# Autodesk Inventor assembly: Bearing Assembly
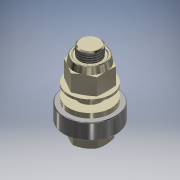
[picture p0: Inventor's stored thumbnail of the model, 180x180]
Saved by Autodesk Inventor 2018.2 (Build 222227000, 227)
## iProperties
Created: 2018-01-21
Part Number: Bearing Assembly
Document SubType Name: Assembly
Designer: torba
Author: torba
## Documents named in this file (6)
- C:\Users\torba\OneDrive\Documents\Inventor\Plasma 5x10\Bearing Assembly.iam
- C:\Users\torba\OneDrive\Documents\Inventor\Plasma 5x10\6202RS Bearing.ipt
- C:\Users\torba\OneDrive\Documents\Inventor\Content Center Files\R2018\en-US\AS 2465(2)\AS 2465 - 9_16 x 1 3_4  UNF.ipt
- C:\Users\torba\OneDrive\Documents\Inventor\Content Center Files\R2018\en-US\ANSI B18.22.1\ANSI B18.22.1 - 9_16 - narrow - Type B.ipt
- C:\Users\torba\OneDrive\Documents\Inventor\Plasma 5x10\Nylock Nut, Inch\Nylock Nut, Inch UNF 9-16.ipt
- C:\Users\torba\OneDrive\Documents\Inventor\Plasma 5x10\Nylock Nut, Inch.ipt
## Components (6 placed, 4 different names)
1. 6202RS Bearing:1 — Mate:1, Mate:5, Mate:7
2. AS 2465 - Inch 9/16 x 1 3/4  UNF:1 — Mate:1, Mate:2, Mate:3, Mate:4, Mate:5, Mate:9
3. Plain Washer (Inch) 9/16 - narrow - Type B:1 — Mate:3, Mate:6, Mate:8
4. Plain Washer (Inch) 9/16 - narrow - Type B:2 — Mate:2, Mate:6, Mate:7
5. Nylock Nut, Inch UNF 9-16:1 — Mate:4, Mate:8, Mate:10
6. Plain Washer (Inch) 9/16 - narrow - Type B:3 — Mate:9, Mate:10
## Relationships (10: Mate 10)
- Mate:1: 6202RS Bearing:1 ↔ AS 2465 - Inch 9/16 x 1 3/4  UNF:1
- Mate:2: AS 2465 - Inch 9/16 x 1 3/4  UNF:1 ↔ Plain Washer (Inch) 9/16 - narrow - Type B:2
- Mate:3: AS 2465 - Inch 9/16 x 1 3/4  UNF:1 ↔ Plain Washer (Inch) 9/16 - narrow - Type B:1
- Mate:4: AS 2465 - Inch 9/16 x 1 3/4  UNF:1 ↔ Nylock Nut, Inch UNF 9-16:1
- Mate:5: 6202RS Bearing:1 ↔ AS 2465 - Inch 9/16 x 1 3/4  UNF:1
- Mate:6: Plain Washer (Inch) 9/16 - narrow - Type B:1 ↔ Plain Washer (Inch) 9/16 - narrow - Type B:2
- Mate:7: 6202RS Bearing:1 ↔ Plain Washer (Inch) 9/16 - narrow - Type B:2
- Mate:8 (7.9502 mm): Plain Washer (Inch) 9/16 - narrow - Type B:1 ↔ Nylock Nut, Inch UNF 9-16:1
- Mate:9: AS 2465 - Inch 9/16 x 1 3/4  UNF:1 ↔ Plain Washer (Inch) 9/16 - narrow - Type B:3
- Mate:10: Nylock Nut, Inch UNF 9-16:1 ↔ Plain Washer (Inch) 9/16 - narrow - Type B:3
